# Autodesk Inventor assembly: WidowX-SOLID
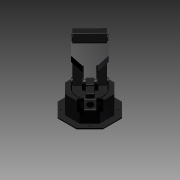
[picture p0: Inventor's stored thumbnail of the model, 180x180]
Saved by Autodesk Inventor 2012 (Build 160160000, 160)
## iProperties
Created: 2013-02-21
Part Number: WidowX-SOLID
Document SubType Name: Assembly
Designer: Andrew
Author: Andrew
## Documents named in this file (8)
- R:\PhantomX Reactor Arm\Reactor_SOLID\Reactor_SOLID.iam
- R:\PhantomX Reactor Arm\Reactor_SOLID\Base.ipt
- R:\PhantomX Reactor Arm\Reactor_SOLID\Shoulder.ipt
- R:\PhantomX Reactor Arm\Reactor_SOLID\Bicep.ipt
- R:\PhantomX Reactor Arm\Reactor_SOLID\ForeArm.ipt
- R:\PhantomX Reactor Arm\Reactor_SOLID\Wrist.ipt
- R:\PhantomX Reactor Arm\Reactor_SOLID\Wrist2.ipt
- R:\PhantomX Reactor Arm\Reactor_SOLID\Imported Components\PX-Gripper\PX-Gripper.iam
## Components (7 placed, 7 different names)
1. Base:1 — Insert:1, Angle:1
2. Shoulder:1 — Insert:1, Insert:7
3. Bicep:1 — Insert:7, Insert:8
4. ForeArm:1 — Insert:8, Insert:9
5. Wrist:1 — Insert:5, Angle:1, Insert:9
6. Wrist2:1 — Insert:5, Insert:6, Angle:2
7. PX-Gripper:1 [sub-assembly] — Insert:6, Angle:2
## Relationships (8: Insert 6, Angle 2)
- Insert:1: Base:1 ↔ Shoulder:1
- Insert:5: Wrist:1 ↔ Wrist2:1
- Angle:1 (0 deg): Base:1 ↔ Wrist:1
- Insert:6: Wrist2:1 ↔ PX-Gripper:1
- Angle:2 (0 deg): Wrist2:1 ↔ PX-Gripper:1
- Insert:7: Shoulder:1 ↔ Bicep:1
- Insert:8: Bicep:1 ↔ ForeArm:1
- Insert:9: ForeArm:1 ↔ Wrist:1
